# Autodesk Inventor assembly: main
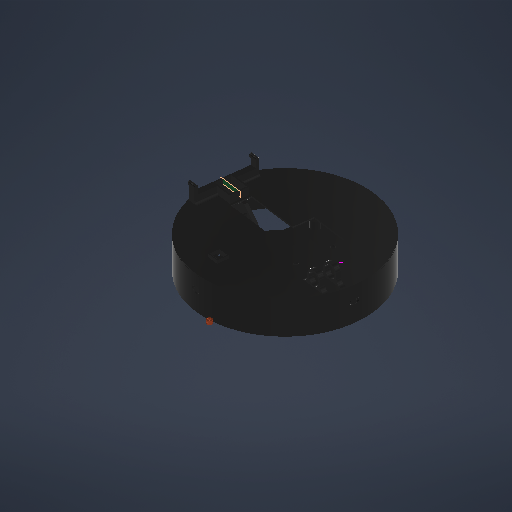
[picture p0: Inventor's stored thumbnail of the model, 512x512]
Saved by Autodesk Inventor 2027 (Build 310192060, 192F)
## iProperties
Created: 2026-04-20
Part Number: main
Document SubType Name: Assembly
Designer: User
Author: User
## Documents named in this file (31)
- C:\Users\Duszy\Desktop\Suntracker\Hardware\Model\main.iam
- C:\Users\Duszy\Desktop\Suntracker\Hardware\Model\Parts\PCB.ipt
- C:\Users\Duszy\Desktop\Suntracker\Hardware\Model\Parts\Middle_part.ipt
- C:\Users\Duszy\Desktop\Suntracker\Hardware\Model\Parts\Top_part.ipt
- C:\Users\Duszy\Desktop\Suntracker\Hardware\Model\Parts\Slip Ring SRM-12-06A\Slip Ring SRM-12-06A\Slip Ring SRM-12-06A.iam
- C:\Users\Duszy\Desktop\Suntracker\Hardware\Model\Parts\Bottom_part.ipt
- C:\Users\Duszy\Desktop\Suntracker\Hardware\Model\Parts\2349K727_Permanently Lubricated Ball Bearing\2349K727_Permanently Lubricated Ball Bearing.ipt
- C:\Users\Duszy\Desktop\Suntracker\Hardware\Model\Parts\N20 DC Gear Motor\N20 DC Gear Motor.ipt
- C:\Users\Duszy\Desktop\Suntracker\Hardware\Model\Parts\pulley_static.ipt
- C:\Users\Duszy\Desktop\Suntracker\Hardware\Model\Parts\pulley_drive.ipt
- C:\Users\Duszy\Desktop\Suntracker\Hardware\Model\Parts\Battery-403040_450mAh\Battery-403040_450mAh.ipt
- C:\Users\Duszy\Desktop\Suntracker\Hardware\Model\Parts\micro usb C Adafruit 4090 - corrected\micro usb C Adafruit 4090 - corrected.ipt
- C:\Users\Duszy\Desktop\Suntracker\Hardware\Model\Parts\LDR\LDR.ipt
- C:\Users\Duszy\Desktop\Suntracker\Hardware\Model\Parts\97048A751_Metric Lead Screw\97048A751_Metric Lead Screw.ipt
- C:\Users\Duszy\Desktop\Suntracker\Hardware\Model\Parts\7487N16_High-Precision Corrosion-Resistant 440C Stainless Steel Ball Bearing\7487N16_High-Precision Corrosion-Resistant 440C Stainless Steel Ball Bearing.ipt
- C:\Users\Duszy\Desktop\Suntracker\Hardware\Model\Parts\konik.ipt
- C:\Users\Duszy\Desktop\Suntracker\Hardware\Model\Parts\link_dom.ipt
- C:\Users\Duszy\Desktop\Suntracker\Hardware\Model\Parts\link_sub.ipt
- C:\Users\Duszy\Desktop\Suntracker\Hardware\Model\Parts\silnik_lock.ipt
- C:\Users\Duszy\Desktop\Suntracker\Hardware\Model\Parts\MicroServo-SG90\MicroServo-SG90.ipt
- C:\Users\Duszy\Desktop\Suntracker\Hardware\Model\Parts\Spur Gear 17 teeth.ipt
- C:\Users\Duszy\Desktop\Suntracker\Hardware\Model\Parts\Spur Gear 30 teeth.ipt
- C:\Users\Duszy\Desktop\Suntracker\Hardware\Model\Parts\flowerstand.ipt
- C:\Users\Duszy\Desktop\Suntracker\Hardware\Model\Parts\7487N13_High-Precision Corrosion-Resistant 440C Stainless Steel Ball Bearing\7487N13_High-Precision Corrosion-Resistant 440C Stainless Steel Ball Bearing.ipt
- C:\Users\Duszy\Desktop\Suntracker\Hardware\Model\Parts\Os_flower.ipt
- C:\Users\Duszy\Desktop\Suntracker\Hardware\Model\Parts\Panel_imitator.iam
- C:\Users\Duszy\Desktop\Suntracker\Hardware\Model\Parts\OS_NORMAL.ipt
- C:\Users\Duszy\Desktop\Suntracker\Hardware\Model\Parts\button 6x6\button 6x6.ipt
- C:\Users\Duszy\Desktop\Suntracker\Hardware\Model\Parts\98886A826_High-Strength High-Temperature PEEK Hex Nut\98886A826_High-Strength High-Temperature PEEK Hex Nut.ipt
- C:\Users\Duszy\Desktop\Suntracker\Hardware\Model\Parts\92000A113_Passivated 18-8 Stainless Steel Pan Head Phillips Screws\92000A113_Passivated 18-8 Stainless Steel Pan Head Phillips Screws.ipt
- C:\Users\Duszy\Desktop\Suntracker\Hardware\Model\Parts\94459A110_Heat-Set Inserts for Plastic\94459A110_Heat-Set Inserts for Plastic.ipt
## Components (54 placed, 30 different names)
1. PCB:1 — Obrotowe:5, Obrotowe:6
2. Middle_part:1 — Obrotowe:5, Obrotowe:18, Obrotowe:19, Sztywne:3, Sztywne:4
3. Top_part:1 — Obrotowe:6, Obrotowe:25, Obrotowe:27, Obrotowe:29, Obrotowe:30, Obrotowe:31, Sztywne:10
4. Slip Ring SRM-12-06A:1 [sub-assembly] — Obrotowe:17, Obrotowe:18, Obrotowe:19, Obrotowe:52
5. Bottom_part:1 — Sztywne:1, Sztywne:2, Obrotowe:15, Obrotowe:16, Obrotowe:17
6. 2349K727_Permanently Lubricated Ball Bearing:1 — Obrotowe:15
7. N20 DC Gear Motor:1 — Obrotowe:9, Sztywne:4
8. pulley_static:1 — Sztywne:1, Obrót:1
9. pulley_drive:1 — Obrotowe:9, Obrót:1
10. micro usb C Adafruit 4090 - corrected:1 — Obrotowe:16
11. 97048A751_Metric Lead Screw:1 — Walcowe:1, Walcowe:2
12. N20 DC Gear Motor:2 — Walcowe:1, Obrotowe:27
13. 7487N16_High-Precision Corrosion-Resistant 440C Stainless Steel Ball Bearing:1 — Obrotowe:21
14. konik:1 — Obrotowe:21, Obrotowe:22, Walcowe:2, Obrotowe:38, Obrotowe:50
15. 7487N16_High-Precision Corrosion-Resistant 440C Stainless Steel Ball Bearing:2 — Obrotowe:22
16. link_dom:1 — Obrotowe:36, Obrotowe:38, Obrotowe:39, Obrotowe:40, Walcowe:3, Sztywne:5
17. link_sub:1 — Obrotowe:28, Walcowe:3
18. 7487N16_High-Precision Corrosion-Resistant 440C Stainless Steel Ball Bearing:3 — Obrotowe:25, Obrotowe:28
19. 7487N16_High-Precision Corrosion-Resistant 440C Stainless Steel Ball Bearing:4 — Obrotowe:29, Obrotowe:49
20. silnik_lock:1 — Obrotowe:30, Obrotowe:31
21. MicroServo-SG90:1 — Obrotowe:32, Obrotowe:36, Obrotowe:39
22. Spur Gear 17 teeth:1 — Obrotowe:33, Obrotowe:40, Obrót:2, Obrotowe:42, Przejściowe:1
23. Spur Gear 30 teeth:1 — Obrotowe:32, Obrót:2
24. 7487N16_High-Precision Corrosion-Resistant 440C Stainless Steel Ball Bearing:5 — Obrotowe:33
25. 7487N13_High-Precision Corrosion-Resistant 440C Stainless Steel Ball Bearing:1 — Obrotowe:41
26. flowerstand:1 — Obrotowe:41, Obrotowe:42, Przejściowe:1, Sztywne:6, Obrotowe:46
27. Os_flower:1 — Sztywne:5
28. Panel_imitator:1 [sub-assembly] — Sztywne:6
29. 7487N13_High-Precision Corrosion-Resistant 440C Stainless Steel Ball Bearing:2 — Obrotowe:46
30. flowerstand:2 — Obrotowe:47
31. Panel_imitator:2 [sub-assembly]
32. 7487N13_High-Precision Corrosion-Resistant 440C Stainless Steel Ball Bearing:3 — Obrotowe:47
33. flowerstand:3 — Obrotowe:48
34. Panel_imitator:3 [sub-assembly]
35. 7487N13_High-Precision Corrosion-Resistant 440C Stainless Steel Ball Bearing:4
36. flowerstand:4 — Obrotowe:48
37. Panel_imitator:4 [sub-assembly]
38. OS_NORMAL:1 — Obrotowe:50
39. OS_NORMAL:2 — Obrotowe:49
40. button 6x6:1 — Sztywne:10
41. 94459A110_Heat-Set Inserts for Plastic:1
42. Battery-403040_450mAh:1 — Sztywne:2
43. Battery-403040_450mAh:2
44. Battery-403040_450mAh:3
45. LDR:1 — Sztywne:3
46. LDR:2
47. LDR:3
48. LDR:4
49. 92000A113_Passivated 18-8 Stainless Steel Pan Head Phillips Screws:1 — Obrotowe:51, Obrotowe:52
50. 98886A826_High-Strength High-Temperature PEEK Hex Nut:1 — Obrotowe:51
51. 92000A113_Passivated 18-8 Stainless Steel Pan Head Phillips Screws:2
52. 98886A826_High-Strength High-Temperature PEEK Hex Nut:2
53. 92000A113_Passivated 18-8 Stainless Steel Pan Head Phillips Screws:3
54. 98886A826_High-Strength High-Temperature PEEK Hex Nut:3
## Component patterns: (3 elements, first: Battery-403040_450mAh:1), (4 elements, first: LDR:1), (3 elements, first: 92000A113_Passivated 18-8 Stainless Steel Pan Head Phillips Screws:1 + 98886A826_High-Strength High-Temperature PEEK Hex Nut:1)
## Relationships (50: RevoluteJoint 34, WeldJoint 10, CylindricalJoint 3, RelateRotation 2, Transitional 1)
- Obrotowe:5 [RevoluteJoint] (-0.1 mm): PCB:1 ↔ Middle_part:1
- Obrotowe:6 [RevoluteJoint] (-0.1 mm): PCB:1 ↔ Top_part:1
- Obrotowe:9 [RevoluteJoint] (1 mm): N20 DC Gear Motor:1 ↔ pulley_drive:1
- Sztywne:1 [WeldJoint]: Bottom_part:1 ↔ pulley_static:1
- Sztywne:2 [WeldJoint] (0.3 mm): Bottom_part:1 ↔ Battery-403040_450mAh:1
- Obrotowe:15 [RevoluteJoint] (-3.1 mm): Bottom_part:1 ↔ 2349K727_Permanently Lubricated Ball Bearing:1
- Obrotowe:16 [RevoluteJoint] (-2.5 mm): Bottom_part:1 ↔ micro usb C Adafruit 4090 - corrected:1
- Obrotowe:17 [RevoluteJoint] (-2.3 mm): Slip Ring SRM-12-06A:1 ↔ Bottom_part:1
- Obrotowe:18 [RevoluteJoint] (-0.2 mm): Middle_part:1 ↔ Slip Ring SRM-12-06A:1
- Obrotowe:19 [RevoluteJoint] (-0.2 mm): Middle_part:1 ↔ Slip Ring SRM-12-06A:1
- Obrót:1 [RelateRotation] (5 ul): pulley_static:1 ↔ pulley_drive:1
- Sztywne:3 [WeldJoint]: Middle_part:1 ↔ LDR:1
- Walcowe:1 [CylindricalJoint]: 97048A751_Metric Lead Screw:1 ↔ N20 DC Gear Motor:2
- Obrotowe:21 [RevoluteJoint] (-2.85 mm): 7487N16_High-Precision Corrosion-Resistant 440C Stainless Steel Ball Bearing:1 ↔ konik:1
- Obrotowe:22 [RevoluteJoint] (-2.85 mm): konik:1 ↔ 7487N16_High-Precision Corrosion-Resistant 440C Stainless Steel Ball Bearing:2
- Obrotowe:25 [RevoluteJoint] (-2.8 mm): Top_part:1 ↔ 7487N16_High-Precision Corrosion-Resistant 440C Stainless Steel Ball Bearing:3
- Obrotowe:27 [RevoluteJoint]: Top_part:1 ↔ N20 DC Gear Motor:2
- Obrotowe:28 [RevoluteJoint] (0.1 mm): link_sub:1 ↔ 7487N16_High-Precision Corrosion-Resistant 440C Stainless Steel Ball Bearing:3
- Walcowe:2 [CylindricalJoint]: 97048A751_Metric Lead Screw:1 ↔ konik:1
- Obrotowe:29 [RevoluteJoint]: Top_part:1 ↔ 7487N16_High-Precision Corrosion-Resistant 440C Stainless Steel Ball Bearing:4
- Obrotowe:30 [RevoluteJoint] (-0.1 mm): Top_part:1 ↔ silnik_lock:1
- Obrotowe:31 [RevoluteJoint] (-0.1 mm): Top_part:1 ↔ silnik_lock:1
- Sztywne:4 [WeldJoint]: Middle_part:1 ↔ N20 DC Gear Motor:1
- Obrotowe:32 [RevoluteJoint]: MicroServo-SG90:1 ↔ Spur Gear 30 teeth:1
- Obrotowe:33 [RevoluteJoint] (-0.23 mm): Spur Gear 17 teeth:1 ↔ 7487N16_High-Precision Corrosion-Resistant 440C Stainless Steel Ball Bearing:5
- Obrotowe:36 [RevoluteJoint]: link_dom:1 ↔ MicroServo-SG90:1
- Obrotowe:38 [RevoluteJoint] (-0.1 mm): konik:1 ↔ link_dom:1
- Obrotowe:39 [RevoluteJoint]: link_dom:1 ↔ MicroServo-SG90:1
- Obrotowe:40 [RevoluteJoint]: link_dom:1 ↔ Spur Gear 17 teeth:1
- Obrót:2 [RelateRotation] (1.7647 ul): Spur Gear 17 teeth:1 ↔ Spur Gear 30 teeth:1
- Obrotowe:41 [RevoluteJoint]: 7487N13_High-Precision Corrosion-Resistant 440C Stainless Steel Ball Bearing:1 ↔ flowerstand:1
- Obrotowe:42 [RevoluteJoint] (0.2 mm): Spur Gear 17 teeth:1 ↔ flowerstand:1
- Przejściowe:1 [Transitional]: Spur Gear 17 teeth:1 ↔ flowerstand:1
- Walcowe:3 [CylindricalJoint]: link_dom:1 ↔ link_sub:1
- Sztywne:5 [WeldJoint] (-1 mm): link_dom:1 ↔ Os_flower:1
- Sztywne:6 [WeldJoint]: flowerstand:1 ↔ Panel_imitator:1
- [RevoluteJoint]: 7487N13_High-Precision Corrosion-Resistant 440C Stainless Steel Ball Bearing:2 ↔ flowerstand:2
- [WeldJoint]: flowerstand:2 ↔ Panel_imitator:2
- [RevoluteJoint]: 7487N13_High-Precision Corrosion-Resistant 440C Stainless Steel Ball Bearing:3 ↔ flowerstand:3
- [WeldJoint]: flowerstand:3 ↔ Panel_imitator:3
- [RevoluteJoint]: 7487N13_High-Precision Corrosion-Resistant 440C Stainless Steel Ball Bearing:4 ↔ flowerstand:4
- [WeldJoint]: flowerstand:4 ↔ Panel_imitator:4
- Obrotowe:46 [RevoluteJoint] (-0.2 mm): flowerstand:1 ↔ 7487N13_High-Precision Corrosion-Resistant 440C Stainless Steel Ball Bearing:2
- Obrotowe:47 [RevoluteJoint] (-0.2 mm): flowerstand:2 ↔ 7487N13_High-Precision Corrosion-Resistant 440C Stainless Steel Ball Bearing:3
- Obrotowe:48 [RevoluteJoint] (-0.2 mm): flowerstand:3 ↔ flowerstand:4
- Obrotowe:49 [RevoluteJoint] (-0.5 mm): 7487N16_High-Precision Corrosion-Resistant 440C Stainless Steel Ball Bearing:4 ↔ OS_NORMAL:2
- Obrotowe:50 [RevoluteJoint] (-0.5 mm): konik:1 ↔ OS_NORMAL:1
- Sztywne:10 [WeldJoint]: Top_part:1 ↔ button 6x6:1
- Obrotowe:51 [RevoluteJoint]: 92000A113_Passivated 18-8 Stainless Steel Pan Head Phillips Screws:1 ↔ 98886A826_High-Strength High-Temperature PEEK Hex Nut:1
- Obrotowe:52 [RevoluteJoint]: Slip Ring SRM-12-06A:1 ↔ 92000A113_Passivated 18-8 Stainless Steel Pan Head Phillips Screws:1
## Named parameters: d417_d372 = 0 mm, d418_d373 = 11.795177 deg, d419_d416 = 0 mm, d420_d372 = 0 mm, d421_d373 = 97.877645 deg, d422_d416 = 0 mm, d423_d372 = 0 mm, d424_d373 = -92.518453 deg, d425_d416 = 0 mm
